# Autodesk Inventor assembly: SansCapacFata
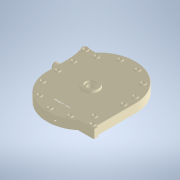
[picture p0: Inventor's stored thumbnail of the model, 180x180]
Saved by Autodesk Inventor 2021 (Build 250183000, 183)
## iProperties
Created: 2021-04-08
Part Number: SansCapacFata
Document SubType Name: Assembly
Designer: Crist
Author: Crist
## Documents named in this file (4)
- C:\Users\Crist\Desktop\Facultate\CAD\#Proiecte\Wankel_GoleaCristian\SansCapacFata.iam
- C:\Users\Crist\Desktop\Facultate\CAD\#Proiecte\Wankel_GoleaCristian\CapacFata.ipt
- C:\Users\Crist\Desktop\Facultate\CAD\#Proiecte\Wankel_GoleaCristian\Pinion.ipt
- C:\Users\Crist\Desktop\Facultate\CAD\#Proiecte\Wankel_GoleaCristian\SubansM4x10.iam
## Components (3 placed, 3 different names)
1. CapacFata:1 — Mate:1, Mate:2, Angle:1
2. Pinion:1 — Mate:1, Mate:2, Angle:1
3. SubansM4x10:1 [sub-assembly]
## Relationships (4: Mate 2, Angle 1, Insert 1)
- Mate:1: CapacFata:1 ↔ Pinion:1
- Mate:2: CapacFata:1 ↔ Pinion:1
- Angle:1 (99 deg): CapacFata:1 ↔ Pinion:1
- [Insert]: Pinion:1 ↔ SubansM4x10:1
